# Autodesk Inventor assembly: Passion-v2
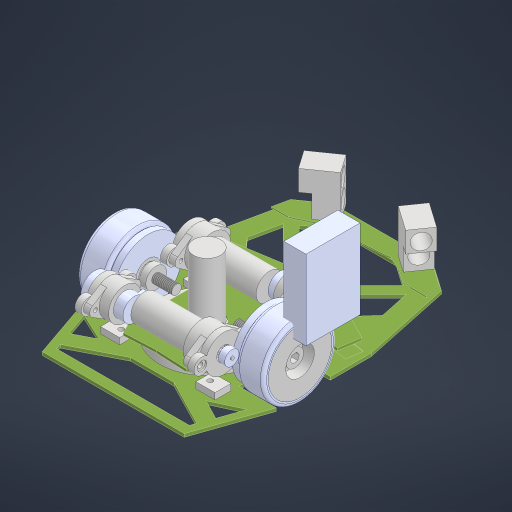
[picture p0: Inventor's stored thumbnail of the model, 512x512]
Saved by Autodesk Inventor 2023.5 (Build 275446000, 446)
## iProperties
Created: 2024-12-07
Part Number: Passion-v2
Document SubType Name: Assembly
Designer: IshiiLabHonda
Author: IshiiLabHonda
## Documents named in this file (21)
- C:\Users\IshiiLabHonda\Documents\Micromouse\Passion-v2\Inventor\Passion-v2.iam
- C:\Users\IshiiLabHonda\Documents\Micromouse\Passion-v2\Inventor\Readymade\Encoder-Gear_M0.3_29T.ipt
- C:\Users\IshiiLabHonda\Documents\Micromouse\Passion-v2\Inventor\Readymade\Encoder-Gear-Spacer.ipt
- C:\Users\IshiiLabHonda\Documents\Micromouse\Passion-v2\Inventor\Readymade\Motor-8523.ipt
- C:\Users\IshiiLabHonda\Documents\Micromouse\Passion-v2\Inventor\Readymade\Pinion-Gear_M0.3_15T.ipt
- C:\Users\IshiiLabHonda\Documents\Micromouse\Passion-v2\Inventor\Readymade\Spur-Gear_M0.3_71T_t2.0_D8.ipt
- C:\Users\IshiiLabHonda\Documents\Micromouse\Passion-v2\Inventor\Readymade\Tire-MZW39-40.ipt
- C:\Users\IshiiLabHonda\Documents\Micromouse\Passion-v2\Inventor\Readymade\Wheel_MZH131W-N2.ipt
- C:\Users\IshiiLabHonda\Documents\Micromouse\Passion-v2\Inventor\Common\spacer_inwheel_1.1.ipt
- C:\Users\IshiiLabHonda\Documents\Micromouse\Passion-v2\Inventor\Common\bearing_SMR63ZZ.ipt
- C:\Users\IshiiLabHonda\Documents\Micromouse\Passion-v2\Inventor\Common\spacer_outwheel_1.6.ipt
- C:\Users\IshiiLabHonda\Documents\Micromouse\Passion-v2\Inventor\Common\M3_bolt.ipt
- C:\Users\IshiiLabHonda\Documents\Micromouse\Passion-v2\Inventor\Readymade\Encoder-7S-400-2MC-50-00E.ipt
- C:\Users\IshiiLabHonda\Documents\Micromouse\Passion-v2\Inventor\Readymade\Motor-8520.ipt
- C:\Users\IshiiLabHonda\Documents\Micromouse\Passion-v2\Inventor\Origin\encoderauxiliary.ipt
- C:\Users\IshiiLabHonda\Documents\Micromouse\Passion-v2\Inventor\Origin\motorauxiliary.ipt
- C:\Users\IshiiLabHonda\Documents\Micromouse\Passion-v2\Inventor\Origin\fan.ipt
- C:\Users\IshiiLabHonda\Documents\Micromouse\Passion-v2\Inventor\Origin\motormount.ipt
- C:\Users\IshiiLabHonda\Documents\Micromouse\Nightfall-Lite_v1\Li-Po_JJRC-150mAh.ipt
- C:\Users\IshiiLabHonda\Documents\Micromouse\Passion-v2\Inventor\Origin\chassis.ipt
- C:\Users\IshiiLabHonda\Documents\Micromouse\Passion-v2\Inventor\Origin\sensorholder_2.ipt
## Components (38 placed, 20 different names)
1. Motor-8520:1 — メイト:35, メイト:39
2. fan:1 — メイト:39, フラッシュ:17
3. Encoder-Gear_M0.3_29T:2
4. Encoder-Gear-Spacer:2
5. Motor-8523:2 — メイト:88
6. Pinion-Gear_M0.3_15T:2
7. Spur-Gear_M0.3_71T_t2.0_D8:2 — 対称度:1
8. Tire-MZW39-40:2
9. Wheel_MZH131W-N2:2
10. spacer_inwheel_1.1:2
11. bearing_SMR63ZZ:3
12. bearing_SMR63ZZ:4
13. spacer_outwheel_1.6:2 — メイト:99
14. M3_bolt:2 — メイト:81, メイト:127
15. Encoder-7S-400-2MC-50-00E:2 — フラッシュ:16, メイト:98, メイト:126
16. encoderauxiliary:2 — フラッシュ:16, メイト:97
17. motorauxiliary:2 — メイト:88, メイト:94, メイト:95, メイト:144
18. motormount:2 — メイト:94, メイト:95, メイト:97, メイト:98, フラッシュ:17, メイト:99, フラッシュ:24, メイト:127, フラッシュ:25, フラッシュ:26, メイト:136, メイト:144
19. Li-Po_JJRC-150mAh:2
20. Encoder-Gear_M0.3_29T:3
21. Encoder-Gear-Spacer:3
22. Motor-8523:3 — メイト:126
23. Pinion-Gear_M0.3_15T:3
24. Spur-Gear_M0.3_71T_t2.0_D8:3 — 対称度:1
25. Tire-MZW39-40:3
26. Wheel_MZH131W-N2:3
27. spacer_inwheel_1.1:3
28. bearing_SMR63ZZ:5
29. bearing_SMR63ZZ:6
30. spacer_outwheel_1.6:3
31. M3_bolt:3 — メイト:128
32. Encoder-7S-400-2MC-50-00E:3
33. encoderauxiliary:3
34. motorauxiliary:3 — メイト:145
35. motormount:3 — フラッシュ:24, メイト:128, フラッシュ:25, フラッシュ:26, メイト:131, メイト:137, メイト:145
36. chassis:1 — メイト:131, フラッシュ:27, メイト:132, フラッシュ:28, メイト:133, メイト:136, メイト:137, メイト:139, メイト:140
37. sensorholder_2:2 — フラッシュ:28, メイト:133, メイト:140
38. sensorholder_2:4 — フラッシュ:27, メイト:132, メイト:139
## Relationships (84: Mate 61, Flush 18, Tangent 4, Symmetry 1)
- メイト:35 [Mate]: Motor-8520:1
- メイト:39 [Mate]: Motor-8520:1 ↔ fan:1
- [Mate]: Encoder-Gear_M0.3_29T:2 ↔ Encoder-Gear-Spacer:2
- [Mate]: Encoder-Gear_M0.3_29T:2 ↔ Encoder-Gear-Spacer:2
- [Mate]: Spur-Gear_M0.3_71T_t2.0_D8:2 ↔ Wheel_MZH131W-N2:2
- [Mate]: Spur-Gear_M0.3_71T_t2.0_D8:2 ↔ Wheel_MZH131W-N2:2
- [Mate]: Tire-MZW39-40:2 ↔ Wheel_MZH131W-N2:2
- [Flush]: Tire-MZW39-40:2 ↔ Wheel_MZH131W-N2:2
- [Mate]: Wheel_MZH131W-N2:2 ↔ bearing_SMR63ZZ:3
- [Mate]: spacer_inwheel_1.1:2 ↔ bearing_SMR63ZZ:3
- [Mate]: bearing_SMR63ZZ:3 ↔ bearing_SMR63ZZ:4
- [Mate]: bearing_SMR63ZZ:3 ↔ spacer_outwheel_1.6:2
- [Mate]: Wheel_MZH131W-N2:2 ↔ M3_bolt:2
- [Mate]: spacer_inwheel_1.1:2 ↔ bearing_SMR63ZZ:4
- [Mate]: spacer_inwheel_1.1:2 ↔ bearing_SMR63ZZ:3
- [Mate]: bearing_SMR63ZZ:4 ↔ M3_bolt:2
- [Flush]: Wheel_MZH131W-N2:2 ↔ bearing_SMR63ZZ:3
- [Mate]: bearing_SMR63ZZ:3 ↔ spacer_outwheel_1.6:2
- [Flush]: Encoder-Gear_M0.3_29T:2 ↔ Spur-Gear_M0.3_71T_t2.0_D8:2
- [Tangent] (0.1 mm): Encoder-Gear_M0.3_29T:2 ↔ Spur-Gear_M0.3_71T_t2.0_D8:2
- [Flush]: Pinion-Gear_M0.3_15T:2 ↔ Spur-Gear_M0.3_71T_t2.0_D8:2
- [Tangent] (0.1 mm): Pinion-Gear_M0.3_15T:2 ↔ Spur-Gear_M0.3_71T_t2.0_D8:2
- [Mate]: Encoder-7S-400-2MC-50-00E:2 ↔ encoderauxiliary:2
- [Flush]: Motor-8523:2 ↔ motorauxiliary:2
- [Mate]: Motor-8523:2 ↔ Pinion-Gear_M0.3_15T:2
- [Mate]: Encoder-Gear-Spacer:2 ↔ Encoder-7S-400-2MC-50-00E:2
- メイト:81 [Mate]: M3_bolt:2
- メイト:88 [Mate]: Motor-8523:2 ↔ motorauxiliary:2
- フラッシュ:16 [Flush]: Encoder-7S-400-2MC-50-00E:2 ↔ encoderauxiliary:2
- メイト:94 [Mate]: motorauxiliary:2 ↔ motormount:2
- メイト:95 [Mate]: motorauxiliary:2 ↔ motormount:2
- メイト:97 [Mate]: encoderauxiliary:2 ↔ motormount:2
- メイト:98 [Mate]: Encoder-7S-400-2MC-50-00E:2 ↔ motormount:2
- フラッシュ:17 [Flush] (-0.5 mm): fan:1 ↔ motormount:2
- メイト:99 [Mate]: spacer_outwheel_1.6:2 ↔ motormount:2
- [Mate]: Encoder-Gear_M0.3_29T:3 ↔ Encoder-Gear-Spacer:3
- [Mate]: Encoder-Gear_M0.3_29T:3 ↔ Encoder-Gear-Spacer:3
- [Mate]: Spur-Gear_M0.3_71T_t2.0_D8:3 ↔ Wheel_MZH131W-N2:3
- [Mate]: Spur-Gear_M0.3_71T_t2.0_D8:3 ↔ Wheel_MZH131W-N2:3
- [Mate]: Tire-MZW39-40:3 ↔ Wheel_MZH131W-N2:3
- [Flush]: Tire-MZW39-40:3 ↔ Wheel_MZH131W-N2:3
- [Mate]: Wheel_MZH131W-N2:3 ↔ bearing_SMR63ZZ:5
- [Mate]: spacer_inwheel_1.1:3 ↔ bearing_SMR63ZZ:5
- [Mate]: bearing_SMR63ZZ:5 ↔ bearing_SMR63ZZ:6
- [Mate]: bearing_SMR63ZZ:5 ↔ spacer_outwheel_1.6:3
- [Mate]: Wheel_MZH131W-N2:3 ↔ M3_bolt:3
- [Mate]: spacer_inwheel_1.1:3 ↔ bearing_SMR63ZZ:6
- [Mate]: spacer_inwheel_1.1:3 ↔ bearing_SMR63ZZ:5
- [Mate]: bearing_SMR63ZZ:6 ↔ M3_bolt:3
- [Flush]: Wheel_MZH131W-N2:3 ↔ bearing_SMR63ZZ:5
- [Mate]: bearing_SMR63ZZ:5 ↔ spacer_outwheel_1.6:3
- [Flush]: Encoder-Gear_M0.3_29T:3 ↔ Spur-Gear_M0.3_71T_t2.0_D8:3
- [Tangent] (0.1 mm): Encoder-Gear_M0.3_29T:3 ↔ Spur-Gear_M0.3_71T_t2.0_D8:3
- [Flush]: Pinion-Gear_M0.3_15T:3 ↔ Spur-Gear_M0.3_71T_t2.0_D8:3
- [Tangent] (0.1 mm): Pinion-Gear_M0.3_15T:3 ↔ Spur-Gear_M0.3_71T_t2.0_D8:3
- [Mate]: Encoder-7S-400-2MC-50-00E:3 ↔ encoderauxiliary:3
- [Flush]: Motor-8523:3 ↔ motorauxiliary:3
- [Mate]: Motor-8523:3 ↔ Pinion-Gear_M0.3_15T:3
- [Mate]: Encoder-Gear-Spacer:3 ↔ Encoder-7S-400-2MC-50-00E:3
- [Mate]: Motor-8523:3 ↔ motorauxiliary:3
- [Flush]: Encoder-7S-400-2MC-50-00E:3 ↔ encoderauxiliary:3
- [Mate]: motorauxiliary:3 ↔ motormount:3
- [Mate]: motorauxiliary:3 ↔ motormount:3
- [Mate]: encoderauxiliary:3 ↔ motormount:3
- [Mate]: Encoder-7S-400-2MC-50-00E:3 ↔ motormount:3
- [Mate]: spacer_outwheel_1.6:3 ↔ motormount:3
- フラッシュ:24 [Flush]: motormount:2 ↔ motormount:3
- メイト:126 [Mate] (1 mm): Encoder-7S-400-2MC-50-00E:2 ↔ Motor-8523:3
- メイト:127 [Mate]: M3_bolt:2 ↔ motormount:2
- メイト:128 [Mate]: M3_bolt:3 ↔ motormount:3
- フラッシュ:25 [Flush]: motormount:2 ↔ motormount:3
- フラッシュ:26 [Flush]: motormount:2 ↔ motormount:3
- 対称度:1 [Symmetry]: Spur-Gear_M0.3_71T_t2.0_D8:2 ↔ Spur-Gear_M0.3_71T_t2.0_D8:3
- メイト:131 [Mate]: motormount:3 ↔ chassis:1
- フラッシュ:27 [Flush]: chassis:1 ↔ sensorholder_2:4
- メイト:132 [Mate]: chassis:1 ↔ sensorholder_2:4
- フラッシュ:28 [Flush]: chassis:1 ↔ sensorholder_2:2
- メイト:133 [Mate]: chassis:1 ↔ sensorholder_2:2
- メイト:136 [Mate]: motormount:2 ↔ chassis:1
- メイト:137 [Mate]: motormount:3 ↔ chassis:1
- メイト:139 [Mate]: chassis:1 ↔ sensorholder_2:4
- メイト:140 [Mate]: chassis:1 ↔ sensorholder_2:2
- メイト:144 [Mate]: motorauxiliary:2 ↔ motormount:2
- メイト:145 [Mate]: motorauxiliary:3 ↔ motormount:3
## Named parameters: d72_d0 = 0 mm, d73_d1 = 0 mm, d74_d2 = 0 mm, d75_d3 = 0 mm, d76_d4 = 0 mm, d77_d5 = 0 mm, d78_d6 = 0 mm, d79_d7 = 0 mm, d80_d8 = 0 mm, d81_d9 = 0 mm, d82_d10 = 0 mm, d83_d11 = 0 mm, d84_d12 = 0 mm, d85_d13 = 0 mm, d86_d14 = 0 mm, d87_d15 = 0 mm, d88_d41 = 0 mm, d89_d42 = 0.1 mm, d90_d43 = 0 mm, d91_d44 = 0.1 mm, d92_d51 = 0 mm, d95_d70 = 0 mm, d96_d71 = 0 mm, d101_d63 = 0 mm, d140_d72_d0 = 0 mm, d141_d73_d1 = 0 mm, d142_d74_d2 = 0 mm, d143_d75_d3 = 0 mm, d144_d76_d4 = 0 mm, d145_d77_d5 = 0 mm, d146_d78_d6 = 0 mm, d147_d79_d7 = 0 mm, d148_d80_d8 = 0 mm, d149_d81_d9 = 0 mm, d150_d82_d10 = 0 mm, d151_d83_d11 = 0 mm, d152_d84_d12 = 0 mm, d153_d85_d13 = 0 mm, d154_d86_d14 = 0 mm, d155_d87_d15 = 0 mm, d156_d88_d41 = 0 mm, d157_d89_d42 = 0.1 mm, d158_d90_d43 = 0 mm, d159_d91_d44 = 0.1 mm, d160_d92_d51 = 0 mm, d161_d95_d70 = 0 mm, d162_d96_d71 = 0 mm, d163_d101_d63 = 0 mm, d164_d120 = 0 mm, d165_d130 = 0 mm, d168_d133 = 0 mm, d169_d134 = 0 mm, d171_d136 = 0 mm, d172_d137 = 0 mm, d173_d139 = 0 mm
